# Autodesk Inventor assembly: RT_FRM_A_Left_Front_Cover
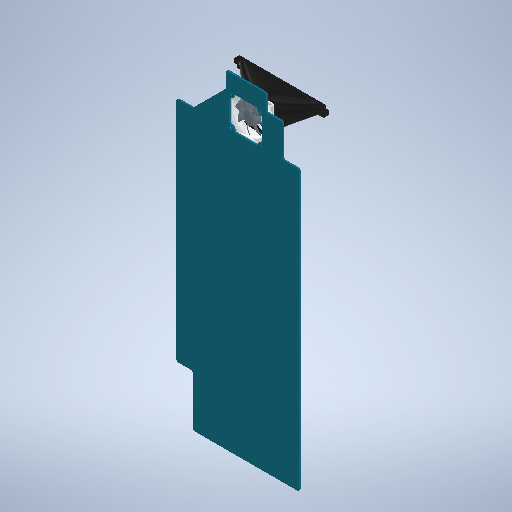
[picture p0: Inventor's stored thumbnail of the model, 512x512]
Saved by Autodesk Inventor 2025.3 (Build 293356000, 356)
## iProperties
Created: 2026-06-07
Part Number: RT_FRM_A_Left_Front_Cover
Document SubType Name: Assembly
Designer: louis
Author: louis
## Documents named in this file (4)
- C:\Users\louis\OneDrive\Desktop\R_Trident\02_CAD\04_Subassemblies\RT_FRM_A_Left_Front_Cover.iam
- C:\Users\louis\OneDrive\Desktop\R_Trident\02_CAD\03_Parts_Custom\RT_FRM_MC_014_FrontCover_L.ipt
- C:\Users\louis\OneDrive\Desktop\R_Trident\02_CAD\03_Parts_Custom\RT_ELE_PR_015_AirDuct.ipt
- C:\Users\louis\OneDrive\Desktop\R_Trident\02_CAD\01_Standard_Parts\04_ELE_Electrical_Automation\NF-R8_Public-CAD\NF-R8_Public-CAD.iam
## Components (3 placed, 3 different names)
1. RT_FRM_MC_014_FrontCover_L:1 — Mate:1, Mate:2, Mate:3, Mate:4, Mate:5
2. RT_ELE_PR_015_AirDuct:1 — Mate:6, Mate:7
3. NF-R8_Public-CAD:1 [sub-assembly] — Mate:3, Mate:4, Mate:5, Mate:6, Mate:7
## Relationships (7: Mate 7)
- Mate:1: RT_FRM_MC_014_FrontCover_L:1
- Mate:2: RT_FRM_MC_014_FrontCover_L:1
- Mate:3: RT_FRM_MC_014_FrontCover_L:1 ↔ NF-R8_Public-CAD:1
- Mate:4: RT_FRM_MC_014_FrontCover_L:1 ↔ NF-R8_Public-CAD:1
- Mate:5: RT_FRM_MC_014_FrontCover_L:1 ↔ NF-R8_Public-CAD:1
- Mate:6: RT_ELE_PR_015_AirDuct:1 ↔ NF-R8_Public-CAD:1
- Mate:7: RT_ELE_PR_015_AirDuct:1 ↔ NF-R8_Public-CAD:1
